# Autodesk Inventor assembly: Shield
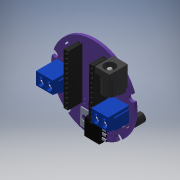
[picture p0: Inventor's stored thumbnail of the model, 180x180]
Saved by Autodesk Inventor 2018 (Build 220112000, 112)
## iProperties
Created: 2017-04-09
Part Number: Shield
Document SubType Name: Assembly
Designer: dkt01
Author: dkt01
## Documents named in this file (8)
- C:\Users\dktur\Dropbox\StackLightMonitor\CAD\Shield.iam
- C:\Users\dktur\Dropbox\StackLightMonitor\CAD\FemaleHeader-02.iam
- C:\Users\dktur\Dropbox\StackLightMonitor\CAD\PCB.ipt
- C:\Users\dktur\Dropbox\StackLightMonitor\CAD\97.ipt
- C:\Users\dktur\Dropbox\StackLightMonitor\CAD\KLDHCX-0202-B_rA2.ipt
- C:\Users\dktur\Dropbox\StackLightMonitor\CAD\Screw Terminal Block 5mm.ipt
- C:\Users\dktur\Dropbox\StackLightMonitor\CAD\LM317.ipt
- C:\Users\dktur\Dropbox\StackLightMonitor\CAD\TO-92.ipt
## Components (11 placed, 7 different names)
1. FemaleHeader-02:1 [sub-assembly] — Mate:2, Tangent:4, Tangent:5, Tangent:8
2. FemaleHeader-02:2 [sub-assembly] — Mate:3, Tangent:9, Tangent:10, Tangent:11
3. PCB:1 — Mate:2, Tangent:4, Tangent:5, Tangent:8, Mate:3, Tangent:9, Tangent:10, Tangent:11, Mate:4, Tangent:12, Tangent:13, Mate:5, Mate:6, Mate:7, Mate:8, Tangent:14, Tangent:15, Mate:9, Tangent:16, Tangent:17, Mate:10, Tangent:18, Tangent:19, Tangent:22, Flush:1, Mate:11, Flush:2, Flush:13, Mate:13, Mate:14
4. 97:1 — Mate:4, Tangent:12, Tangent:13
5. KLDHCX-0202-B_rA2:1 — Mate:5, Mate:6, Mate:7
6. Screw Terminal Block 5mm:1 — Mate:8, Tangent:14, Tangent:15
7. Screw Terminal Block 5mm:2 — Mate:9, Tangent:16, Tangent:17
8. LM317:1 — Mate:10, Tangent:18, Tangent:19
9. TO-92:1 — Flush:13, Mate:13
10. TO-92:2 — Flush:2, Mate:14
11. TO-92:3 — Tangent:22, Flush:1, Mate:11
## Relationships (30: Tangent 15, Mate 12, Flush 3)
- Mate:2: FemaleHeader-02:1 ↔ PCB:1
- Tangent:4: FemaleHeader-02:1 ↔ PCB:1
- Tangent:5: FemaleHeader-02:1 ↔ PCB:1
- Tangent:8: FemaleHeader-02:1 ↔ PCB:1
- Mate:3: FemaleHeader-02:2 ↔ PCB:1
- Tangent:9: FemaleHeader-02:2 ↔ PCB:1
- Tangent:10: FemaleHeader-02:2 ↔ PCB:1
- Tangent:11: FemaleHeader-02:2 ↔ PCB:1
- Mate:4: PCB:1 ↔ 97:1
- Tangent:12: PCB:1 ↔ 97:1
- Tangent:13: PCB:1 ↔ 97:1
- Mate:5: PCB:1 ↔ KLDHCX-0202-B_rA2:1
- Mate:6: PCB:1 ↔ KLDHCX-0202-B_rA2:1
- Mate:7: PCB:1 ↔ KLDHCX-0202-B_rA2:1
- Mate:8: PCB:1 ↔ Screw Terminal Block 5mm:1
- Tangent:14: PCB:1 ↔ Screw Terminal Block 5mm:1
- Tangent:15: PCB:1 ↔ Screw Terminal Block 5mm:1
- Mate:9: PCB:1 ↔ Screw Terminal Block 5mm:2
- Tangent:16: PCB:1 ↔ Screw Terminal Block 5mm:2
- Tangent:17: PCB:1 ↔ Screw Terminal Block 5mm:2
- Mate:10: PCB:1 ↔ LM317:1
- Tangent:18: PCB:1 ↔ LM317:1
- Tangent:19: PCB:1 ↔ LM317:1
- Tangent:22: PCB:1 ↔ TO-92:3
- Flush:1 (1 mm): PCB:1 ↔ TO-92:3
- Mate:11: PCB:1 ↔ TO-92:3
- Flush:2 (-1 mm): PCB:1 ↔ TO-92:2
- Flush:13 (-1 mm): PCB:1 ↔ TO-92:1
- Mate:13: PCB:1 ↔ TO-92:1
- Mate:14: PCB:1 ↔ TO-92:2
